# Autodesk Inventor assembly: Sand Timer
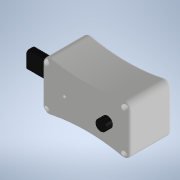
[picture p0: Inventor's stored thumbnail of the model, 180x180]
Saved by Autodesk Inventor 2021 (Build 250183000, 183)
## iProperties
Created: 2024-02-01
Part Number: Sand Timer
Document SubType Name: Assembly
Designer: maxsm
Author: maxsm
## Documents named in this file (10)
- C:\Users\maxsm\root\SandTimer\v2\casings\Sand Timer.iam
- C:\Users\maxsm\root\SandTimer\v2\casings\Controller Board.ipt
- C:\Users\maxsm\root\SandTimer\v2\casings\16-Pin Header.ipt
- C:\Users\maxsm\root\SandTimer\v2\casings\12-Pin Header.ipt
- C:\Users\maxsm\root\SandTimer\v2\casings\LED Board.ipt
- C:\Users\maxsm\root\SandTimer\v2\casings\Battery.ipt
- C:\Users\maxsm\root\SandTimer\v2\casings\Bottom.ipt
- C:\Users\maxsm\root\SandTimer\v2\casings\USB C Plug.ipt
- C:\Users\maxsm\root\SandTimer\v2\casings\Top.ipt
- C:\Users\maxsm\OneDrive\Documents\Inventor\Content Center Files\R2021\en-US\ANSI B18.6.7M(02)\ANSI B18.6.7M - M2.5x0.45 x 6(6).ipt
## Components (12 placed, 9 different names)
1. Controller Board:1 — Mate:1, Mate:2, Mate:3, Mate:4, Mate:5, Mate:6, Mate:10, Flush:1, Flush:2, Mate:11, Mate:12, Mate:13, Mate:14, Mate:15, Flush:3, Mate:21, Mate:23, Mate:25, Mate:27
2. 16-Pin Header:1 — Mate:1, Mate:2, Mate:3, Mate:7, Mate:8, Mate:9
3. 12-Pin Header:1 — Mate:4, Mate:5, Mate:6
4. LED Board:1 — Mate:7, Mate:8, Mate:9
5. Battery:1 — Mate:10, Flush:1, Flush:2
6. Bottom:1 — Mate:11, Mate:12, Mate:13, Mate:17, Mate:22, Mate:24, Mate:26, Mate:28, Mate:29, Mate:30
7. USB C Plug:1 — Mate:14, Mate:15, Flush:3
8. Top:1 — Mate:17, Mate:29, Mate:30
9. Square Recessed Pan Head Machine Screw - Type III - Metric M2.5x0.45 x 6:1 — Mate:21, Mate:22
10. Square Recessed Pan Head Machine Screw - Type III - Metric M2.5x0.45 x 6:2 — Mate:23, Mate:24
11. Square Recessed Pan Head Machine Screw - Type III - Metric M2.5x0.45 x 6:3 — Mate:25, Mate:26
12. Square Recessed Pan Head Machine Screw - Type III - Metric M2.5x0.45 x 6:4 — Mate:27, Mate:28
## Relationships (29: Mate 26, Flush 3)
- Mate:1: Controller Board:1 ↔ 16-Pin Header:1
- Mate:2: Controller Board:1 ↔ 16-Pin Header:1
- Mate:3: Controller Board:1 ↔ 16-Pin Header:1
- Mate:4: Controller Board:1 ↔ 12-Pin Header:1
- Mate:5: Controller Board:1 ↔ 12-Pin Header:1
- Mate:6: Controller Board:1 ↔ 12-Pin Header:1
- Mate:7: 16-Pin Header:1 ↔ LED Board:1
- Mate:8: 16-Pin Header:1 ↔ LED Board:1
- Mate:9: 16-Pin Header:1 ↔ LED Board:1
- Mate:10 (2 mm): Controller Board:1 ↔ Battery:1
- Flush:1 (-3 mm): Controller Board:1 ↔ Battery:1
- Flush:2: Controller Board:1 ↔ Battery:1
- Mate:11: Controller Board:1 ↔ Bottom:1
- Mate:12: Controller Board:1 ↔ Bottom:1
- Mate:13: Controller Board:1 ↔ Bottom:1
- Mate:14: Controller Board:1 ↔ USB C Plug:1
- Mate:15: Controller Board:1 ↔ USB C Plug:1
- Flush:3 (1.5 mm): Controller Board:1 ↔ USB C Plug:1
- Mate:17: Bottom:1 ↔ Top:1
- Mate:21: Controller Board:1 ↔ Square Recessed Pan Head Machine Screw - Type III - Metric M2.5x0.45 x 6:1
- Mate:22: Bottom:1 ↔ Square Recessed Pan Head Machine Screw - Type III - Metric M2.5x0.45 x 6:1
- Mate:23: Controller Board:1 ↔ Square Recessed Pan Head Machine Screw - Type III - Metric M2.5x0.45 x 6:2
- Mate:24: Bottom:1 ↔ Square Recessed Pan Head Machine Screw - Type III - Metric M2.5x0.45 x 6:2
- Mate:25: Controller Board:1 ↔ Square Recessed Pan Head Machine Screw - Type III - Metric M2.5x0.45 x 6:3
- Mate:26: Bottom:1 ↔ Square Recessed Pan Head Machine Screw - Type III - Metric M2.5x0.45 x 6:3
- Mate:27: Controller Board:1 ↔ Square Recessed Pan Head Machine Screw - Type III - Metric M2.5x0.45 x 6:4
- Mate:28: Bottom:1 ↔ Square Recessed Pan Head Machine Screw - Type III - Metric M2.5x0.45 x 6:4
- Mate:29: Bottom:1 ↔ Top:1
- Mate:30: Bottom:1 ↔ Top:1
